# Autodesk Inventor assembly: F_Foot
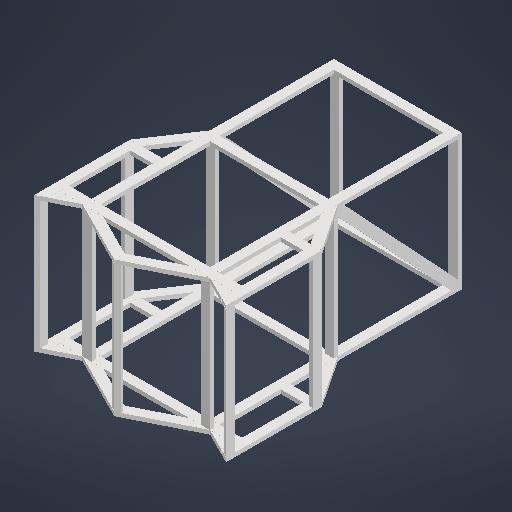
[picture p0: Inventor's stored thumbnail of the model, 512x512]
Saved by Autodesk Inventor 2026 (Build 300175000, 175)
## iProperties
Created: 2025-09-08
Part Number: F_Foot
Document SubType Name: Assembly
Designer: trott
Author: trott
## Documents named in this file (13)
- C:\Users\trott\Documents\UofSC-ASME-Tiger-Burn-Design-2025\CAD\Legs\Front Foot\F_Foot.iam
- C:\Users\trott\Documents\UofSC-ASME-Tiger-Burn-Design-2025\CAD\Legs\Front Foot\2x4x48.ipt
- C:\Users\trott\Documents\UofSC-ASME-Tiger-Burn-Design-2025\CAD\Legs\Front Foot\2x4x41.ipt
- C:\Users\trott\Documents\UofSC-ASME-Tiger-Burn-Design-2025\CAD\Legs\Front Foot\2x4x65.ipt
- C:\Users\trott\Documents\UofSC-ASME-Tiger-Burn-Design-2025\CAD\Legs\Front Foot\2x4x8.5.ipt
- C:\Users\trott\Documents\UofSC-ASME-Tiger-Burn-Design-2025\CAD\Legs\Front Foot\S_2x4x36.ipt
- C:\Users\trott\Documents\UofSC-ASME-Tiger-Burn-Design-2025\CAD\Legs\Front Foot\S_2x4x9.503.ipt
- C:\Users\trott\Documents\UofSC-ASME-Tiger-Burn-Design-2025\CAD\Legs\Front Foot\S_2x4x26.833.ipt
- C:\Users\trott\Documents\UofSC-ASME-Tiger-Burn-Design-2025\CAD\Legs\Front Foot\S2_2x4x48.ipt
- C:\Users\trott\Documents\UofSC-ASME-Tiger-Burn-Design-2025\CAD\Legs\Front Foot\S_2x4x48.ipt
- C:\Users\trott\Documents\UofSC-ASME-Tiger-Burn-Design-2025\CAD\Legs\Front Foot\S_2x4x21.633.ipt
- C:\Users\trott\Documents\UofSC-ASME-Tiger-Burn-Design-2025\CAD\Legs\Front Foot\2x4x91.ipt
- C:\Users\trott\Documents\UofSC-ASME-Tiger-Burn-Design-2025\CAD\Legs\Front Foot\S_2x4x65.795.ipt
## Components (43 placed, 12 different names)
1. 2x4x48:7 — Mate:17, Flush:23, Flush:24
2. 2x4x48:8 — Mate:18, Flush:25, Flush:26
3. S2_2x4x48:1 — Mate:19, Flush:27, Flush:28
4. S_2x4x48:1
5. S_2x4x48:2
6. 2x4x41:3 — Flush:41
7. 2x4x41:4 — Mate:30, Flush:43, Flush:44
8. 2x4x48:9 — Mate:32, Flush:49, Mate:33, Mate:39
9. 2x4x48:10 — Mate:34, Flush:50, Mate:35, Mate:36
10. S_2x4x65.795:1 — Mate:36, Mate:37, Flush:51
11. S_2x4x65.795:2 — Mate:38, Mate:39, Flush:52
12. 2x4x48:2 — Flush:31, Flush:41, Flush:43
13. 2x4x48:3
14. 2x4x48:4 — Mate:20
15. 2x4x48:5 — Flush:32, Mate:22, Flush:33
16. S_2x4x21.633:1
17. S_2x4x21.633:2
18. S_2x4x21.633:3
19. S_2x4x21.633:4 — Mate:20, Flush:29
20. 2x4x91:1 — Mate:21, Flush:30, Flush:31, Mate:30, Flush:44, Flush:46, Flush:47, Mate:34, Flush:50, Mate:35, Mate:37, Flush:51
21. 2x4x91:2 — Mate:23, Flush:33, Flush:34, Mate:31, Flush:45, Flush:48, Mate:32, Flush:49, Mate:33, Mate:38, Flush:52
22. 2x4x41:5 — Mate:31, Flush:45, Flush:46, Flush:47, Flush:48
23. 2x4x8.5:2 — Flush:16
24. S_2x4x36:2 — Mate:7, Flush:15, Flush:16, Mate:10, Flush:18, Mate:18, Flush:25, Flush:26, Flush:29
25. 2x4x65:1 — Mate:6, Flush:13, Mate:7, Flush:15, Mate:9, Mate:11, Mate:12, Flush:19, Mate:15, Flush:20, Mate:21, Flush:30, Flush:32, Mate:23, Flush:34
26. S_2x4x9.503:2 — Mate:10, Mate:11, Flush:18, Mate:22
27. S_2x4x26.833:2 — Mate:14, Mate:15, Flush:20, Flush:27
28. S_2x4x26.833:1 — Mate:12, Mate:13, Flush:19, Mate:14, Mate:19, Flush:28
29. S_2x4x9.503:1 — Mate:8, Flush:17, Mate:9, Mate:13
30. S_2x4x36:1 — Mate:6, Flush:13, Flush:14, Mate:8, Flush:17, Mate:17, Flush:23, Flush:24
31. 2x4x8.5:1 — Flush:14
32. 2x4x91:3
33. 2x4x91:4
34. 2x4x41:6
35. 2x4x8.5:3
36. S_2x4x36:3
37. 2x4x65:2
38. S_2x4x9.503:3
39. S_2x4x26.833:3
40. S_2x4x26.833:4
41. S_2x4x9.503:4
42. S_2x4x36:4
43. 2x4x8.5:4
## Component patterns: (4 elements, first: 2x4x48:2), (2 elements, first: S_2x4x21.633:1 + S_2x4x21.633:2), (2 elements, first: 2x4x91:1 + 2x4x91:2 + 2x4x41:5 + 2x4x8.5:2 + S_2x4x36:2 + 2x4x65:1 + S_2x4x9.503:2 + S_2x4x26.833:2 + S_2x4x26.833:1 + S_2x4x9.503:1 + S_2x4x36:1 + 2x4x8.5:1)
## Relationships (58: Flush 31, Mate 27)
- Mate:6: 2x4x65:1 ↔ S_2x4x36:1
- Flush:13: 2x4x65:1 ↔ S_2x4x36:1
- Flush:14: S_2x4x36:1 ↔ 2x4x8.5:1
- Mate:7: S_2x4x36:2 ↔ 2x4x65:1
- Flush:15: S_2x4x36:2 ↔ 2x4x65:1
- Flush:16: 2x4x8.5:2 ↔ S_2x4x36:2
- Mate:8: S_2x4x9.503:1 ↔ S_2x4x36:1
- Flush:17: S_2x4x9.503:1 ↔ S_2x4x36:1
- Mate:9: 2x4x65:1 ↔ S_2x4x9.503:1
- Mate:10: S_2x4x36:2 ↔ S_2x4x9.503:2
- Mate:11: 2x4x65:1 ↔ S_2x4x9.503:2
- Flush:18: S_2x4x36:2 ↔ S_2x4x9.503:2
- Mate:12: 2x4x65:1 ↔ S_2x4x26.833:1
- Mate:13: S_2x4x26.833:1 ↔ S_2x4x9.503:1
- Flush:19: 2x4x65:1 ↔ S_2x4x26.833:1
- Mate:14: S_2x4x26.833:2 ↔ S_2x4x26.833:1
- Mate:15: 2x4x65:1 ↔ S_2x4x26.833:2
- Flush:20: 2x4x65:1 ↔ S_2x4x26.833:2
- Mate:17: 2x4x48:7 ↔ S_2x4x36:1
- Flush:23: 2x4x48:7 ↔ S_2x4x36:1
- Flush:24: 2x4x48:7 ↔ S_2x4x36:1
- Mate:18: 2x4x48:8 ↔ S_2x4x36:2
- Flush:25: 2x4x48:8 ↔ S_2x4x36:2
- Flush:26: 2x4x48:8 ↔ S_2x4x36:2
- Mate:19: S2_2x4x48:1 ↔ S_2x4x26.833:1
- Flush:27: S2_2x4x48:1 ↔ S_2x4x26.833:2
- Flush:28: S2_2x4x48:1 ↔ S_2x4x26.833:1
- Mate:20: 2x4x48:4 ↔ S_2x4x21.633:4
- Flush:29: S_2x4x21.633:4 ↔ S_2x4x36:2
- Mate:21: 2x4x91:1 ↔ 2x4x65:1
- Flush:30: 2x4x91:1 ↔ 2x4x65:1
- Flush:31: 2x4x48:2 ↔ 2x4x91:1
- Flush:32: 2x4x48:5 ↔ 2x4x65:1
- Mate:22: 2x4x48:5 ↔ S_2x4x9.503:2
- Mate:23: 2x4x91:2 ↔ 2x4x65:1
- Flush:33: 2x4x48:5 ↔ 2x4x91:2
- Flush:34: 2x4x91:2 ↔ 2x4x65:1
- Flush:41: 2x4x41:3 ↔ 2x4x48:2
- Mate:30: 2x4x41:4 ↔ 2x4x91:1
- Flush:43: 2x4x41:4 ↔ 2x4x48:2
- Flush:44: 2x4x41:4 ↔ 2x4x91:1
- Mate:31: 2x4x91:2 ↔ 2x4x41:5
- Flush:45: 2x4x91:2 ↔ 2x4x41:5
- Flush:46: 2x4x91:1 ↔ 2x4x41:5
- Flush:47: 2x4x91:1 ↔ 2x4x41:5
- Flush:48: 2x4x91:2 ↔ 2x4x41:5
- Mate:32: 2x4x48:9 ↔ 2x4x91:2
- Flush:49: 2x4x48:9 ↔ 2x4x91:2
- Mate:33: 2x4x48:9 ↔ 2x4x91:2
- Mate:34: 2x4x48:10 ↔ 2x4x91:1
- Flush:50: 2x4x48:10 ↔ 2x4x91:1
- Mate:35: 2x4x48:10 ↔ 2x4x91:1
- Mate:36: 2x4x48:10 ↔ S_2x4x65.795:1
- Mate:37: S_2x4x65.795:1 ↔ 2x4x91:1
- Flush:51: S_2x4x65.795:1 ↔ 2x4x91:1
- Mate:38: S_2x4x65.795:2 ↔ 2x4x91:2
- Mate:39: 2x4x48:9 ↔ S_2x4x65.795:2
- Flush:52: S_2x4x65.795:2 ↔ 2x4x91:2
